# Autodesk Inventor assembly: CombinedPiHolder
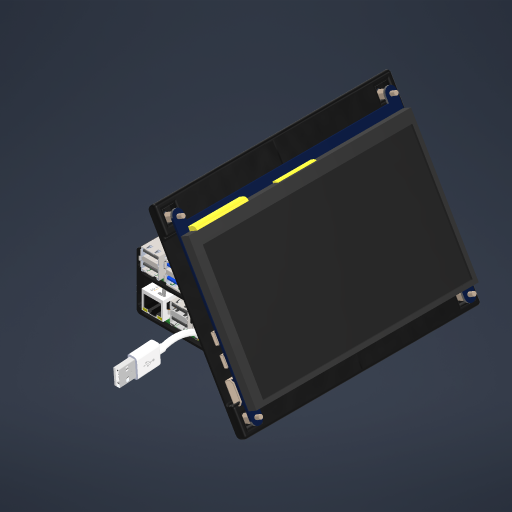
[picture p0: Inventor's stored thumbnail of the model, 512x512]
Saved by Autodesk Inventor 2023 (Build 270158000, 158)
## iProperties
Created: 2023-02-13
Part Number: CombinedPiHolder
Document SubType Name: Assembly
Designer: uzair
Mass: 272.337 g
Surface Area: 1385.92 cm^2
Volume: 272.337 cm^3
Density: 1 g/cm^3
Author: uzair
## Documents named in this file (11)
- C:\Users\uzair\Programming\Capstone-MJ02\documentation\3D Models\CombinedPiHolder.iam
- C:\Users\uzair\Programming\Capstone-MJ02\documentation\3D Models\Raspberry_Pi_4_Sleeve_v1-0_MAIN.ipt
- C:\Users\uzair\Programming\Capstone-MJ02\documentation\3D Models\Raspberry_Pi_B+_Sleeve_v2-1_MAIN.ipt
- C:\Users\uzair\Programming\Capstone-MJ02\documentation\3D Models\UE306_Sleeve.ipt
- C:\Users\uzair\Downloads\raspberry-pi-4-model-b-1.snapshot.3\Raspberry Pi 4 Model B.iam
- C:\Users\uzair\Downloads\usb-0-to-fast-ethernet-adapter-1.snapshot.1\USB Etherent Adapter\Part1.ipt
- C:\Users\uzair\Downloads\raspberry-pi-3-model-b-reference-design-solidworks-cad-rpi-raspberrypi-raspberry-pi-1.snapshot.83\Exported Versions\Raspberry Pi 3 Light Version.ipt
- C:\Users\uzair\Downloads\noctua-nf-a4x10-2.snapshot.1\Noctua-NF-A4x10.ipt
- C:\Users\uzair\Programming\Capstone-MJ02\documentation\3D Models\CombinedScreenHolder.iam
- C:\Users\uzair\Downloads\hdmi-raspberry-pi-touch-screen-1024-600-7inch-model-1.snapshot.3\lcd 7inch cap 1024 600.ipt
- C:\Users\uzair\Downloads\ettinger-standoff-nickel-plated-brass-m-f-m2-m8-1.snapshot.2\stp M3\Abstandzbolzen Messing vernickelt I-A M3_-_Ettinger - 5.13.083 (M3x8).ipt
## Components (13 placed, 10 different names)
1. Raspberry_Pi_4_Sleeve_v1-0_MAIN:1 — Mate:1, Mate:2, Mate:3, Mate:4, Mate:7, Mate:8, Mate:15, Mate:16, Mate:17
2. Raspberry_Pi_B+_Sleeve_v2-1_MAIN:1 — Mate:1, Mate:2, Mate:12, Mate:13, Mate:14
3. UE306_Sleeve:1 — Mate:3, Mate:4, Mate:9, Mate:10, Mate:11, Mate:18, Mate:19
4. Raspberry Pi 4 Model B:1 [sub-assembly] — Mate:15, Mate:16, Mate:17
5. Part1:1 — Mate:9, Mate:10, Mate:11
6. Raspberry Pi 3 Light Version:1 — Mate:12, Mate:13, Mate:14
7. Noctua-NF-A4x10:1 — Mate:7, Mate:8
8. CombinedScreenHolder:1 [sub-assembly] — Mate:18, Mate:19, Mate:24
9. lcd 7inch cap 1024 600:1 — Mate:20, Mate:21, Mate:22, Mate:23
10. Abstandzbolzen Messing vernickelt I-A M3_-_Ettinger - 5.13.083 (M3x8):4 — Mate:20
11. Abstandzbolzen Messing vernickelt I-A M3_-_Ettinger - 5.13.083 (M3x8):5 — Mate:23, Mate:24
12. Abstandzbolzen Messing vernickelt I-A M3_-_Ettinger - 5.13.083 (M3x8):6 — Mate:22
13. Abstandzbolzen Messing vernickelt I-A M3_-_Ettinger - 5.13.083 (M3x8):7 — Mate:21
## Relationships (22: Mate 22)
- Mate:1: Raspberry_Pi_4_Sleeve_v1-0_MAIN:1 ↔ Raspberry_Pi_B+_Sleeve_v2-1_MAIN:1
- Mate:2: Raspberry_Pi_4_Sleeve_v1-0_MAIN:1 ↔ Raspberry_Pi_B+_Sleeve_v2-1_MAIN:1
- Mate:3: Raspberry_Pi_4_Sleeve_v1-0_MAIN:1 ↔ UE306_Sleeve:1
- Mate:4: Raspberry_Pi_4_Sleeve_v1-0_MAIN:1 ↔ UE306_Sleeve:1
- Mate:7: Raspberry_Pi_4_Sleeve_v1-0_MAIN:1 ↔ Noctua-NF-A4x10:1
- Mate:8: Raspberry_Pi_4_Sleeve_v1-0_MAIN:1 ↔ Noctua-NF-A4x10:1
- Mate:9: UE306_Sleeve:1 ↔ Part1:1
- Mate:10: UE306_Sleeve:1 ↔ Part1:1
- Mate:11: UE306_Sleeve:1 ↔ Part1:1
- Mate:12: Raspberry_Pi_B+_Sleeve_v2-1_MAIN:1 ↔ Raspberry Pi 3 Light Version:1
- Mate:13: Raspberry_Pi_B+_Sleeve_v2-1_MAIN:1 ↔ Raspberry Pi 3 Light Version:1
- Mate:14: Raspberry_Pi_B+_Sleeve_v2-1_MAIN:1 ↔ Raspberry Pi 3 Light Version:1
- Mate:15: Raspberry_Pi_4_Sleeve_v1-0_MAIN:1 ↔ Raspberry Pi 4 Model B:1
- Mate:16: Raspberry_Pi_4_Sleeve_v1-0_MAIN:1 ↔ Raspberry Pi 4 Model B:1
- Mate:17: Raspberry_Pi_4_Sleeve_v1-0_MAIN:1 ↔ Raspberry Pi 4 Model B:1
- Mate:18: UE306_Sleeve:1 ↔ CombinedScreenHolder:1
- Mate:19: UE306_Sleeve:1 ↔ CombinedScreenHolder:1
- Mate:20: lcd 7inch cap 1024 600:1 ↔ Abstandzbolzen Messing vernickelt I-A M3_-_Ettinger - 5.13.083 (M3x8):4
- Mate:21: lcd 7inch cap 1024 600:1 ↔ Abstandzbolzen Messing vernickelt I-A M3_-_Ettinger - 5.13.083 (M3x8):7
- Mate:22: lcd 7inch cap 1024 600:1 ↔ Abstandzbolzen Messing vernickelt I-A M3_-_Ettinger - 5.13.083 (M3x8):6
- Mate:23: lcd 7inch cap 1024 600:1 ↔ Abstandzbolzen Messing vernickelt I-A M3_-_Ettinger - 5.13.083 (M3x8):5
- Mate:24: CombinedScreenHolder:1 ↔ Abstandzbolzen Messing vernickelt I-A M3_-_Ettinger - 5.13.083 (M3x8):5
